# Autodesk Inventor assembly: EDM Middle Shield New
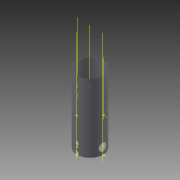
[picture p0: Inventor's stored thumbnail of the model, 180x180]
Saved by Autodesk Inventor 2015 (Build 190159000, 159)
## iProperties
Created: 2014-07-11
Part Number: EDM Middle Shield New
Document SubType Name: Assembly
Designer: I Rabey
Author: I Rabey
## Documents named in this file (5)
- C:\ColdMatter\CADFiles\EDM Machine\EDM Middle Shield\EDM Middle Shield New.iam
- C:\ColdMatter\CADFiles\EDM Machine\EDM Middle Shield\Lower Front Half 2014 Replacement.ipt
- C:\ColdMatter\CADFiles\EDM Machine\EDM Middle Shield\Lower Back Half 2014 Replacement.ipt
- C:\ColdMatter\CADFiles\EDM Machine\EDM Middle Shield\Upper Front Half 2014 Replacement.ipt
- C:\ColdMatter\CADFiles\EDM Machine\EDM Middle Shield\Upper Back Half 2014 Replacement.ipt
## Components (4 placed, 4 different names)
1. Lower Front Half 2014 Replacement:1 — Mate:1, Mate:2, Mate:3, Mate:4, Mate:5, Mate:7
2. Lower Back Half 2014 Replacement:1 — Mate:3, Mate:4, Mate:5, Mate:6, Mate:10
3. Upper Front Half 2014 Replacement:1 — Mate:9, Mate:10, Mate:11
4. Upper Back Half 2014 Replacement:1 — Mate:6, Mate:7, Mate:8, Mate:9, Mate:11
## Relationships (11: Mate 11)
- Mate:1: Lower Front Half 2014 Replacement:1
- Mate:2: Lower Front Half 2014 Replacement:1
- Mate:3: Lower Front Half 2014 Replacement:1 ↔ Lower Back Half 2014 Replacement:1
- Mate:4: Lower Front Half 2014 Replacement:1 ↔ Lower Back Half 2014 Replacement:1
- Mate:5: Lower Front Half 2014 Replacement:1 ↔ Lower Back Half 2014 Replacement:1
- Mate:6: Lower Back Half 2014 Replacement:1 ↔ Upper Back Half 2014 Replacement:1
- Mate:7: Lower Front Half 2014 Replacement:1 ↔ Upper Back Half 2014 Replacement:1
- Mate:8: Upper Back Half 2014 Replacement:1
- Mate:9: Upper Front Half 2014 Replacement:1 ↔ Upper Back Half 2014 Replacement:1
- Mate:10: Lower Back Half 2014 Replacement:1 ↔ Upper Front Half 2014 Replacement:1
- Mate:11: Upper Front Half 2014 Replacement:1 ↔ Upper Back Half 2014 Replacement:1
